# Autodesk Inventor assembly: jubilee_snapshot_mar_16_2020
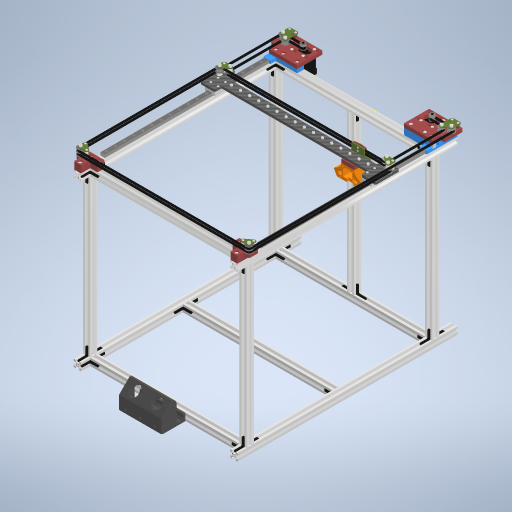
[picture p0: Inventor's stored thumbnail of the model, 512x512]
Saved by Autodesk Inventor 2024.2 (Build 282272000, 272)
## iProperties
Created: 2020-03-16
Part Number: jubilee_snapshot_mar_16_2020
Description: STEP AP203
Document SubType Name: Assembly
Designer: Micha
Sending System: SolidWorks 2019
Preprocessor: SwSTEP 2.0
Title: jubilee_snapshot_mar_16_2020.STEP
Revision Number: ANY
## Documents named in this file (6)
- C:\Users\Micha\Documents\493\claw\cad\Inventor\claw_machine.iam
- C:\Users\Micha\Documents\493\claw\cad\Inventor\lower_frame_assembly.iam
- C:\Users\Micha\Documents\493\claw\cad\Inventor\jubilee_xy_frame_assembly.iam
- C:\Users\Micha\Documents\493\claw\cad\Inventor\330mm_2020_tslot_extrusion.ipt
- C:\Users\Micha\Documents\493\claw\cad\Inventor\build_plate_assembly.iam
- C:\Users\Micha\Documents\493\claw\cad\Inventor\joystick_mount.ipt
## Components (9 placed, 9 different names)
1. lower_frame_assembly_1 [sub-assembly] — Mate:1, Flush:1, Mate:2, Flush:2
2. jubilee_xy_frame_assembly_2 [sub-assembly]
3. 330mm_2020_tslot_extrusion_6
4. 330mm_2020_tslot_extrusion_7
5. 330mm_2020_tslot_extrusion_8 — Mate:3
6. 330mm_2020_tslot_extrusion_9
7. build_plate_assembly_13 [sub-assembly]
8. joystick_mount:1 — Mate:1, Flush:1
9. 330mm_2020_tslot_extrusion:5 — Mate:2, Flush:2, Mate:3
## Relationships (5: Mate 3, Flush 2)
- Mate:1: lower_frame_assembly_1 ↔ joystick_mount:1
- Flush:1: lower_frame_assembly_1 ↔ joystick_mount:1
- Mate:2: lower_frame_assembly_1 ↔ 330mm_2020_tslot_extrusion:5
- Flush:2: lower_frame_assembly_1 ↔ 330mm_2020_tslot_extrusion:5
- Mate:3 (194.5 mm): 330mm_2020_tslot_extrusion_8 ↔ 330mm_2020_tslot_extrusion:5
